# Autodesk Inventor assembly: ASY MSC 900.1 BASE FRAME
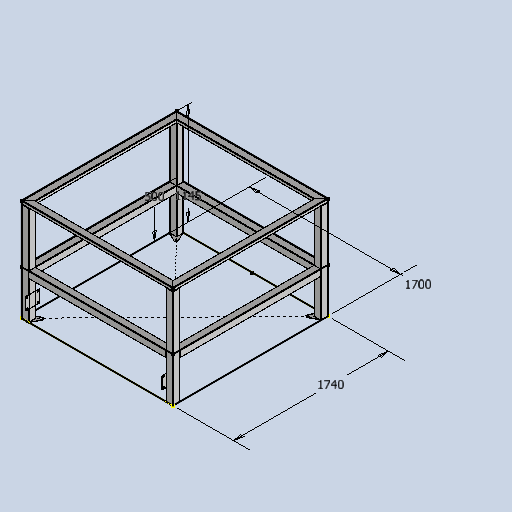
[picture p0: Inventor's stored thumbnail of the model, 512x512]
Saved by Autodesk Inventor 2025 (Build 290162010, 162A)
## iProperties
Created: 2024-05-19
Part Number: ASY MSC 900.1 BASE FRAME
Document SubType Name: Assembly
Designer: admin
Stock Number: МОО 900.1 стол
_SolveAssemblyDoc: Frame Generator Solve Assembly
_Version: 15.0.0
Author: admin
## Documents named in this file (5)
- C:\Users\admin\YandexDisk-badmisterfox\домашниий пк\Inventor\Manturovo\Manturovo_Se-clar\ASY MSC 900.1 base frame.iam
- C:\Users\admin\YandexDisk-badmisterfox\домашниий пк\Inventor\Manturovo\Manturovo_Se-clar\MSC DIM 009.1 base frame sketch.ipt
- C:\Users\admin\YandexDisk-badmisterfox\домашниий пк\Inventor\Manturovo\Manturovo_Se-clar\Pillars\ASY MSC 900.1.1 base frame.iam
- C:\Users\admin\YandexDisk-badmisterfox\домашниий пк\Inventor\Manturovo\Manturovo_Se-clar\MSC 901 base plate.ipt
- C:\Users\admin\YandexDisk-badmisterfox\домашниий пк\Inventor\Manturovo\Manturovo_Se-clar\MSC 908 transverse pillar plate.ipt
## Components (8 placed, 4 different names)
1. MSC DIM 009.1 base frame sketch.ipt:1
2. ASY MSC 900.1.1 base frame.iam:1 [sub-assembly] — Rigid:1, Rigid:2, Rigid:3, Rigid:4, Mate:1, Flush:1, Mate:3
3. MSC 901 base plate.ipt:1 — Rigid:2
4. MSC 901 base plate.ipt:2 — Rigid:1
5. MSC 901 base plate.ipt:3 — Rigid:4
6. MSC 901 base plate.ipt:4 — Rigid:3, Mate:2
7. MSC 908 transverse pillar plate:1 — Mate:1, Mate:2, Flush:1, Flush:2, Flush:3
8. MSC 908 transverse pillar plate:2 — Mate:3, Flush:2, Flush:3
## Relationships (10: WeldJoint 4, Mate 3, Flush 3)
- Rigid:1 [WeldJoint]: ASY MSC 900.1.1 base frame.iam:1 ↔ MSC 901 base plate.ipt:2
- Rigid:2 [WeldJoint]: ASY MSC 900.1.1 base frame.iam:1 ↔ MSC 901 base plate.ipt:1
- Rigid:3 [WeldJoint]: ASY MSC 900.1.1 base frame.iam:1 ↔ MSC 901 base plate.ipt:4
- Rigid:4 [WeldJoint]: ASY MSC 900.1.1 base frame.iam:1 ↔ MSC 901 base plate.ipt:3
- Mate:1: ASY MSC 900.1.1 base frame.iam:1 ↔ MSC 908 transverse pillar plate:1
- Mate:2 (130 mm): MSC 901 base plate.ipt:4 ↔ MSC 908 transverse pillar plate:1
- Flush:1 (-40 mm): ASY MSC 900.1.1 base frame.iam:1 ↔ MSC 908 transverse pillar plate:1
- Mate:3: ASY MSC 900.1.1 base frame.iam:1 ↔ MSC 908 transverse pillar plate:2
- Flush:2: MSC 908 transverse pillar plate:1 ↔ MSC 908 transverse pillar plate:2
- Flush:3: MSC 908 transverse pillar plate:1 ↔ MSC 908 transverse pillar plate:2
